# Autodesk Inventor assembly: сборка серва 45_ЗЕРКАЛО2
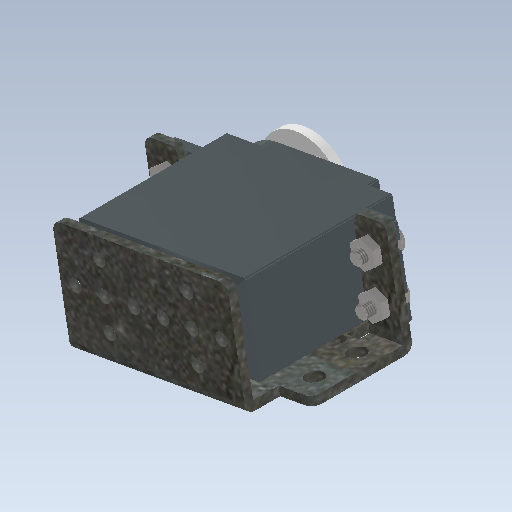
[picture p0: Inventor's stored thumbnail of the model, 512x512]
Saved by Autodesk Inventor 2020.1 (Build 241239000, 239)
## iProperties
Created: 2021-08-12
Part Number: сборка серва 45_ЗЕРКАЛО2
Document SubType Name: Assembly
Designer: User
Author: User
## Documents named in this file (6)
- D:\GitHub\avatar-kvantoriada\3D\сборка серва 45_ЗЕРКАЛО2.iam
- D:\GitHub\avatar-kvantoriada\3D\Деталь4_ЗЕРКАЛО3.ipt
- D:\GitHub\avatar-kvantoriada\3D\MG996R_ЗЕРКАЛО3.ipt
- D:\GitHub\avatar-kvantoriada\3D\Деталь5_ЗЕРКАЛО3.ipt
- C:\Users\User\Documents\Inventor\Content Center Files\R2020\ru-RU\AS 1427(08)\AS 1427 - M3 x 8(6) I.ipt
- C:\Users\User\Documents\Inventor\Content Center Files\R2020\ru-RU\AS 1474(1)\AS 1474 - M3(1).ipt
## Components (12 placed, 5 different names)
1. Деталь4_ЗЕРКАЛО3:1 — Жесткий:1, Жесткий:8, Жесткий:7, Жесткий:6, Жесткий:9
2. MG996R_ЗЕРКАЛО3:1 — Совмещение:2, Совмещение:1, Жесткий:1, Жесткий:3, Жесткий:2, Жесткий:5, Жесткий:4
3. Деталь5_ЗЕРКАЛО3:1 — Совмещение:2, Совмещение:1, Жесткий:13
4. AS 1427 Z - метрическая M3 x 8:1 — Жесткий:3
5. AS 1427 Z - метрическая M3 x 8:2 — Жесткий:2
6. AS 1427 Z - метрическая M3 x 8:3 — Жесткий:5
7. AS 1427 Z - метрическая M3 x 8:4 — Жесткий:4
8. AS 1474 - метрическая M3:1 — Жесткий:8
9. AS 1474 - метрическая M3:2 — Жесткий:7
10. AS 1474 - метрическая M3:3 — Жесткий:6
11. AS 1474 - метрическая M3:4 — Жесткий:9
12. AS 1427 Z - метрическая M3 x 8:5 — Жесткий:13
## Relationships (12: WeldJoint 10, Mate 2)
- Совмещение:2 [Mate]: MG996R_ЗЕРКАЛО3:1 ↔ Деталь5_ЗЕРКАЛО3:1
- Совмещение:1 [Mate]: MG996R_ЗЕРКАЛО3:1 ↔ Деталь5_ЗЕРКАЛО3:1
- Жесткий:1 [WeldJoint]: Деталь4_ЗЕРКАЛО3:1 ↔ MG996R_ЗЕРКАЛО3:1
- Жесткий:3 [WeldJoint]: MG996R_ЗЕРКАЛО3:1 ↔ AS 1427 Z - метрическая M3 x 8:1
- Жесткий:2 [WeldJoint]: MG996R_ЗЕРКАЛО3:1 ↔ AS 1427 Z - метрическая M3 x 8:2
- Жесткий:5 [WeldJoint]: MG996R_ЗЕРКАЛО3:1 ↔ AS 1427 Z - метрическая M3 x 8:3
- Жесткий:4 [WeldJoint]: MG996R_ЗЕРКАЛО3:1 ↔ AS 1427 Z - метрическая M3 x 8:4
- Жесткий:8 [WeldJoint]: Деталь4_ЗЕРКАЛО3:1 ↔ AS 1474 - метрическая M3:1
- Жесткий:7 [WeldJoint]: Деталь4_ЗЕРКАЛО3:1 ↔ AS 1474 - метрическая M3:2
- Жесткий:6 [WeldJoint]: Деталь4_ЗЕРКАЛО3:1 ↔ AS 1474 - метрическая M3:3
- Жесткий:9 [WeldJoint]: Деталь4_ЗЕРКАЛО3:1 ↔ AS 1474 - метрическая M3:4
- Жесткий:13 [WeldJoint]: Деталь5_ЗЕРКАЛО3:1 ↔ AS 1427 Z - метрическая M3 x 8:5
